# Autodesk Inventor assembly: HDzero microi assy
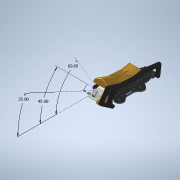
[picture p0: Inventor's stored thumbnail of the model, 180x180]
Saved by Autodesk Inventor 2020 (Build 240168000, 168)
## iProperties
Created: 2022-05-03
Part Number: HDzero microi assy
Document SubType Name: Assembly
Designer: Steven
Author: Steven
## Documents named in this file (8)
- Y:\FPV drone stuff\0 Street League\Frames\PB-Kauri-X\3D prints\35 mm canopy\work in progress prints\HDzero microi assy.iam
- Y:\FPV drone stuff\0 Street League\Frames\PB-Kauri-X\Kauri side plate.ipt
- Y:\FPV drone stuff\0 Street League\Frames\PB-Kauri-X\3D prints\35 mm canopy\KauriCanopy Pb.ipt
- Y:\FPV drone stuff\0 Street League\Frames\PB-Kauri-X\Kauri mid plate v2.ipt
- Y:\FPV drone stuff\0 Street League\Frames\PB-Kauri-X\3D prints\35 mm canopy\KauriFrontLink 35mm.ipt
- Y:\FPV drone stuff\0 Street League\Frames\PB-Kauri-X\3D prints\35 mm canopy\KauriRearLink 35mm no brass insert.ipt
- Y:\FPV drone stuff\0 Street League\Frames\PB-Kauri-X\3D prints\35 mm canopy\35mm standoff.ipt
- Y:\FPV drone stuff\0 Street League\Frames\PB-Kauri-X\3D prints\35 mm canopy\work in progress prints\modular predator mount.iam
## Components (9 placed, 7 different names)
1. Kauri side plate:1 — Insert:2, Insert:4, Insert:5, Insert:6, Mate:4
2. Kauri side plate:2 — Insert:1, Insert:3, Insert:9, Insert:10, Mate:3
3. KauriCanopy Pb:1 — Insert:1, Insert:2, Insert:3, Insert:4
4. KauriFrontLink 35mm:1 — Insert:5, Flush:1, Mate:1, Insert:7
5. KauriRearLink 35mm no brass insert:1 — Insert:6, Flush:1, Insert:8
6. Kauri mid plate v2:1 — Mate:1, Insert:7, Insert:8, Mate:7
7. 35mm standoff:1 — Insert:9, Mate:6
8. 35mm standoff:2 — Insert:10, Mate:5
9. modular predator mount:1 [sub-assembly] — Mate:4, Mate:5, Mate:6
## Relationships (17: Insert 10, Mate 6, Flush 1)
- Insert:1: Kauri side plate:2 ↔ KauriCanopy Pb:1
- Insert:2: Kauri side plate:1 ↔ KauriCanopy Pb:1
- Insert:3: Kauri side plate:2 ↔ KauriCanopy Pb:1
- Insert:4: Kauri side plate:1 ↔ KauriCanopy Pb:1
- Insert:5: Kauri side plate:1 ↔ KauriFrontLink 35mm:1
- Insert:6: Kauri side plate:1 ↔ KauriRearLink 35mm no brass insert:1
- Flush:1: KauriFrontLink 35mm:1 ↔ KauriRearLink 35mm no brass insert:1
- Mate:1: KauriFrontLink 35mm:1 ↔ Kauri mid plate v2:1
- Insert:7: KauriFrontLink 35mm:1 ↔ Kauri mid plate v2:1
- Insert:8: KauriRearLink 35mm no brass insert:1 ↔ Kauri mid plate v2:1
- Insert:9: Kauri side plate:2 ↔ 35mm standoff:1
- Insert:10: Kauri side plate:2 ↔ 35mm standoff:2
- Mate:3: Kauri side plate:2
- Mate:4 (6.4 mm): Kauri side plate:1 ↔ modular predator mount:1
- Mate:5: 35mm standoff:2 ↔ modular predator mount:1
- Mate:6: 35mm standoff:1 ↔ modular predator mount:1
- Mate:7: Kauri mid plate v2:1
